# Autodesk Inventor assembly: Hybrid
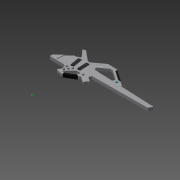
[picture p0: Inventor's stored thumbnail of the model, 180x180]
Saved by Autodesk Inventor 2020.4 (Build 244396010, 396A)
## iProperties
Created: 2022-11-11
Part Number: Hybrid
Document SubType Name: Assembly
Designer: valer
Author: valer
## Documents named in this file (6)
- C:\Users\Val\Desktop\hybrid\src\Hybrid.iam
- C:\Users\Val\Desktop\hybrid\src\Hybrid.ipt
- C:\Users\Val\Desktop\hybrid\src\01BinaryLogo.ipt
- C:\Users\Val\Desktop\hybrid\src\OscilloscopeScreen.ipt
- C:\Users\Val\Desktop\hybrid\src\BottomGrip.ipt
- C:\Users\Val\Desktop\hybrid\src\TopGrip.ipt
## Components (5 placed, 5 different names)
1. Hybrid:1 — Flush:2, Mate:2, Mate:3, Mate:4, Mate:5, Mate:6, Mate:7, Mate:8, Mate:9, Mate:10, Mate:11, Mate:12
2. 01BinaryLogo:1 — Mate:4, Mate:5, Mate:6
3. OscilloscopeScreen:1 — Flush:2, Mate:2, Mate:3
4. BottomGrip:1 — Mate:7, Mate:8, Mate:9
5. TopGrip:1 — Mate:10, Mate:11, Mate:12
## Relationships (12: Mate 11, Flush 1)
- Flush:2: Hybrid:1 ↔ OscilloscopeScreen:1
- Mate:2: Hybrid:1 ↔ OscilloscopeScreen:1
- Mate:3: Hybrid:1 ↔ OscilloscopeScreen:1
- Mate:4: Hybrid:1 ↔ 01BinaryLogo:1
- Mate:5: Hybrid:1 ↔ 01BinaryLogo:1
- Mate:6: Hybrid:1 ↔ 01BinaryLogo:1
- Mate:7: Hybrid:1 ↔ BottomGrip:1
- Mate:8: Hybrid:1 ↔ BottomGrip:1
- Mate:9: Hybrid:1 ↔ BottomGrip:1
- Mate:10: Hybrid:1 ↔ TopGrip:1
- Mate:11: Hybrid:1 ↔ TopGrip:1
- Mate:12: Hybrid:1 ↔ TopGrip:1
